# Autodesk Inventor assembly: Assembly
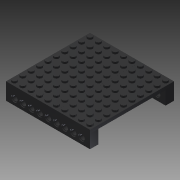
[picture p0: Inventor's stored thumbnail of the model, 180x180]
Saved by Autodesk Inventor 2013 (Build 170138000, 138)
## iProperties
Created: 2013-06-01
Part Number: Assembly
Document SubType Name: Assembly
Designer: Masta
Author: Masta
## Documents named in this file (8)
- D:\work\Legoduino\3D\Assembly.iam
- D:\work\Legoduino\3D\LEGO Plate 4x10.ipt
- D:\work\Legoduino\3D\LEGO Technic Brick 1x8 with Holes.ipt
- D:\work\Legoduino\3D\LEGO Technic Brick 1x10 with Holes.ipt
- D:\work\Legoduino\3D\LEGO Stud 1x1 Transparent Dark Blue.ipt
- D:\work\Legoduino\3D\LEGO Plate 1x10.ipt
- D:\work\Legoduino\3D\LEGO Stud 1x1 Transparent Green.ipt
- D:\work\Legoduino\3D\LEGO Plate 6x10.ipt
## Components (9 placed, 7 different names)
1. LEGO Plate 4x10:2 — Insert:7, Insert:8, Insert:9, Insert:16
2. LEGO Technic Brick 1x8 with Holes:1 — Insert:13, Insert:14, Flush:1, Flush:2, Mate:1
3. LEGO Technic Brick 1x10 with Holes:1 — Insert:3, Insert:4, Mate:2, Mate:3
4. LEGO Technic Brick 1x10 with Holes:2 — Insert:1, Insert:2
5. LEGO Stud 1x1 Transparent Dark Blue:1 — Insert:13, Insert:19, Flush:1
6. LEGO Plate 1x10:1 — Insert:3, Insert:4, Insert:7, Insert:8, Insert:15
7. LEGO Plate 1x10:2 — Insert:1, Insert:2, Insert:9, Insert:16, Insert:17
8. LEGO Stud 1x1 Transparent Green:1 — Insert:14, Insert:18, Flush:2
9. LEGO Plate 6x10:1 — Insert:15, Insert:17, Insert:18, Insert:19
## Relationships (19: Insert 14, Mate 3, Flush 2)
- Insert:1: LEGO Technic Brick 1x10 with Holes:2 ↔ LEGO Plate 1x10:2
- Insert:2: LEGO Technic Brick 1x10 with Holes:2 ↔ LEGO Plate 1x10:2
- Insert:3: LEGO Technic Brick 1x10 with Holes:1 ↔ LEGO Plate 1x10:1
- Insert:4: LEGO Technic Brick 1x10 with Holes:1 ↔ LEGO Plate 1x10:1
- Insert:7: LEGO Plate 4x10:2 ↔ LEGO Plate 1x10:1
- Insert:8: LEGO Plate 4x10:2 ↔ LEGO Plate 1x10:1
- Insert:9: LEGO Plate 4x10:2 ↔ LEGO Plate 1x10:2
- Insert:13: LEGO Technic Brick 1x8 with Holes:1 ↔ LEGO Stud 1x1 Transparent Dark Blue:1
- Insert:14: LEGO Technic Brick 1x8 with Holes:1 ↔ LEGO Stud 1x1 Transparent Green:1
- Insert:15: LEGO Plate 1x10:1 ↔ LEGO Plate 6x10:1
- Insert:16: LEGO Plate 4x10:2 ↔ LEGO Plate 1x10:2
- Insert:17: LEGO Plate 1x10:2 ↔ LEGO Plate 6x10:1
- Insert:18: LEGO Stud 1x1 Transparent Green:1 ↔ LEGO Plate 6x10:1
- Insert:19: LEGO Stud 1x1 Transparent Dark Blue:1 ↔ LEGO Plate 6x10:1
- Flush:1: LEGO Technic Brick 1x8 with Holes:1 ↔ LEGO Stud 1x1 Transparent Dark Blue:1
- Flush:2: LEGO Technic Brick 1x8 with Holes:1 ↔ LEGO Stud 1x1 Transparent Green:1
- Mate:1: LEGO Technic Brick 1x8 with Holes:1
- Mate:2: LEGO Technic Brick 1x10 with Holes:1
- Mate:3: LEGO Technic Brick 1x10 with Holes:1
